# Autodesk Inventor assembly: BaseAssembly
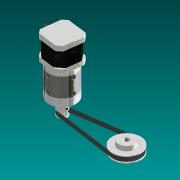
[picture p0: Inventor's stored thumbnail of the model, 180x180]
Saved by Autodesk Inventor 2020.2 (Build 242310000, 310)
## iProperties
Created: 2020-05-14
Part Number: BaseAssembly
Document SubType Name: Assembly
Designer: Svend
Author: Svend
## Documents named in this file (6)
- C:\Users\Svend\OneDrive\Documents\GitHub\BeerMinder\3D-model\Base (Axis 1)\BaseAssembly.iam
- C:\Users\Svend\OneDrive\Documents\GitHub\BeerMinder\3D-model\Nema17MetGearbox.iam
- C:\Users\Svend\OneDrive\Documents\GitHub\BeerMinder\3D-model\pulleys\GT2 Timing Pulley 20T - 8mm as.ipt
- C:\Users\Svend\OneDrive\Documents\GitHub\BeerMinder\3D-model\pulleys\GT2 Timing Pulley 60T - 8mm as.ipt
- C:\Users\Svend\OneDrive\Documents\Inventor\Content Center Files\R2020\en-US\ISO 4026\ISO 4026 - M4 x 8 - ISO.ipt
- C:\Users\Svend\OneDrive\Documents\GitHub\BeerMinder\3D-model\pulleys\Tandriem20naar60T.ipt
## Components (6 placed, 5 different names)
1. Nema17MetGearbox:1 [sub-assembly] — Mate:1, Flush:1
2. GT2 Timing Pulley 20T - 8mm as:1 — Mate:1, Flush:1, Flush:2, Mate:7
3. GT2 Timing Pulley 60T - 8mm as:1 — Flush:2, Mate:2, Mate:3, Mate:4, Mate:5, Mate:6, Mate:8
4. ISO 4026 M4 x 8:1 — Mate:3, Mate:5
5. ISO 4026 M4 x 8:2 — Mate:2, Mate:4
6. Tandriem20naar60T:1 — Mate:6, Mate:7, Mate:8
## Relationships (10: Mate 8, Flush 2)
- Mate:1: Nema17MetGearbox:1 ↔ GT2 Timing Pulley 20T - 8mm as:1
- Flush:1: Nema17MetGearbox:1 ↔ GT2 Timing Pulley 20T - 8mm as:1
- Flush:2: GT2 Timing Pulley 20T - 8mm as:1 ↔ GT2 Timing Pulley 60T - 8mm as:1
- Mate:2: GT2 Timing Pulley 60T - 8mm as:1 ↔ ISO 4026 M4 x 8:2
- Mate:3: GT2 Timing Pulley 60T - 8mm as:1 ↔ ISO 4026 M4 x 8:1
- Mate:4 (-12.5 mm): GT2 Timing Pulley 60T - 8mm as:1 ↔ ISO 4026 M4 x 8:2
- Mate:5 (-12.5 mm): GT2 Timing Pulley 60T - 8mm as:1 ↔ ISO 4026 M4 x 8:1
- Mate:6: GT2 Timing Pulley 60T - 8mm as:1 ↔ Tandriem20naar60T:1
- Mate:7: GT2 Timing Pulley 20T - 8mm as:1 ↔ Tandriem20naar60T:1
- Mate:8 (0.5 mm): GT2 Timing Pulley 60T - 8mm as:1 ↔ Tandriem20naar60T:1
